# Autodesk Inventor assembly: assembly
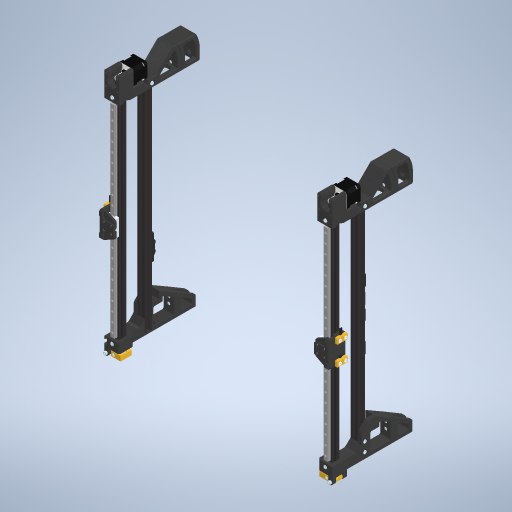
[picture p0: Inventor's stored thumbnail of the model, 512x512]
Saved by Autodesk Inventor 2024 (Build 280153020, 153B)
## iProperties
Created: 2023-11-07
Part Number: assembly
Description: FreeCAD Model
Document SubType Name: Assembly
Designer: torban
Authority: Unknown
Sending System: FreeCAD
Preprocessor: Open CASCADE STEP processor 7.6
Title: Open CASCADE Shape Model
Author: Author
## Documents named in this file (149)
- D:\GIT\lumenpnp\pnp\cad\STEP\Y-Gantry\Y-Gantry.iam
- D:\GIT\lumenpnp\pnp\cad\STEP\Y-Gantry\extrusion-cable-clip002.ipt
- D:\GIT\lumenpnp\pnp\cad\STEP\Y-Gantry\Y-Gantry-Left.iam
- D:\GIT\lumenpnp\pnp\cad\STEP\Y-Gantry\Back-Right-Leg.iam
- D:\GIT\lumenpnp\pnp\cad\STEP\Y-Gantry\Front-Right-Leg.iam
- D:\GIT\lumenpnp\pnp\cad\STEP\Y-Gantry\Y-Gantry-Right-Linear-Rail.iam
- D:\GIT\lumenpnp\pnp\cad\STEP\Y-Gantry\Y-Gantry-Slider-Right.iam
- D:\GIT\lumenpnp\pnp\cad\STEP\Y-Gantry\extrusion-cable-clip003.ipt
- D:\GIT\lumenpnp\pnp\cad\STEP\Y-Gantry\extrusion-cable-clip001.ipt
- D:\GIT\lumenpnp\pnp\cad\STEP\Y-Gantry\extrusion-cable-clip.ipt
- D:\GIT\lumenpnp\pnp\cad\STEP\Y-Gantry\vslot-extrusion-20mmx20mmx600mm001.ipt
- D:\GIT\lumenpnp\pnp\cad\STEP\Y-Gantry\vslot-extrusion-20mmx20mmx600mm002.ipt
- D:\GIT\lumenpnp\pnp\cad\STEP\Y-Gantry\GT2-pulley003.ipt
- D:\GIT\lumenpnp\pnp\cad\STEP\Y-Gantry\M3x8-Screw466.ipt
- D:\GIT\lumenpnp\pnp\cad\STEP\Y-Gantry\M3x8-Screw467.ipt
- D:\GIT\lumenpnp\pnp\cad\STEP\Y-Gantry\M3x8-Screw468.ipt
- D:\GIT\lumenpnp\pnp\cad\STEP\Y-Gantry\M3x8-Screw469.ipt
- D:\GIT\lumenpnp\pnp\cad\STEP\Y-Gantry\NEMA17-stepper004.ipt
- D:\GIT\lumenpnp\pnp\cad\STEP\Y-Gantry\M5x10-Screw345.ipt
- D:\GIT\lumenpnp\pnp\cad\STEP\Y-Gantry\M5x10-Screw346.ipt
- D:\GIT\lumenpnp\pnp\cad\STEP\Y-Gantry\M5x10-Screw347.ipt
- D:\GIT\lumenpnp\pnp\cad\STEP\Y-Gantry\M5-tslot-nut013.ipt
- D:\GIT\lumenpnp\pnp\cad\STEP\Y-Gantry\M5-tslot-nut014.ipt
- D:\GIT\lumenpnp\pnp\cad\STEP\Y-Gantry\M5-tslot-nut015.ipt
- D:\GIT\lumenpnp\pnp\cad\STEP\Y-Gantry\back-leg.ipt
- D:\GIT\lumenpnp\pnp\cad\STEP\Y-Gantry\Back-Right-Leg-Extension.iam
- D:\GIT\lumenpnp\pnp\cad\STEP\Y-Gantry\back-leg-extension_001.ipt
- D:\GIT\lumenpnp\pnp\cad\STEP\Y-Gantry\M5-Nut1086.ipt
- D:\GIT\lumenpnp\pnp\cad\STEP\Y-Gantry\M5x16-Screw219.ipt
- D:\GIT\lumenpnp\pnp\cad\STEP\Y-Gantry\M5-tslot-nut008.ipt
- D:\GIT\lumenpnp\pnp\cad\STEP\Y-Gantry\GT2-idler003.ipt
- D:\GIT\lumenpnp\pnp\cad\STEP\Y-Gantry\M5-Nut627.ipt
- D:\GIT\lumenpnp\pnp\cad\STEP\Y-Gantry\M5x25-Screw128.ipt
- D:\GIT\lumenpnp\pnp\cad\STEP\Y-Gantry\M5-Nut628.ipt
- D:\GIT\lumenpnp\pnp\cad\STEP\Y-Gantry\M3x16-Screw086.ipt
- D:\GIT\lumenpnp\pnp\cad\STEP\Y-Gantry\M3-Nut465.ipt
- D:\GIT\lumenpnp\pnp\cad\STEP\Y-Gantry\M5x10-Screw338.ipt
- D:\GIT\lumenpnp\pnp\cad\STEP\Y-Gantry\M5x10-Screw339.ipt
- D:\GIT\lumenpnp\pnp\cad\STEP\Y-Gantry\M5x10-Screw340.ipt
- D:\GIT\lumenpnp\pnp\cad\STEP\Y-Gantry\M5-tslot-nut007.ipt
- D:\GIT\lumenpnp\pnp\cad\STEP\Y-Gantry\M3-cap-nut.ipt
- D:\GIT\lumenpnp\pnp\cad\STEP\Y-Gantry\M5-tslot-nut009.ipt
- D:\GIT\lumenpnp\pnp\cad\STEP\Y-Gantry\M5x40-Screw345.ipt
- D:\GIT\lumenpnp\pnp\cad\STEP\Y-Gantry\y2-belt-tension-arm.ipt
- D:\GIT\lumenpnp\pnp\cad\STEP\Y-Gantry\front-right-leg.ipt
- D:\GIT\lumenpnp\pnp\cad\STEP\Y-Gantry\Front-Right-Leg-Extension.iam
- D:\GIT\lumenpnp\pnp\cad\STEP\Y-Gantry\M5x16-Screw222.ipt
- D:\GIT\lumenpnp\pnp\cad\STEP\Y-Gantry\M5x16-Screw221.ipt
- D:\GIT\lumenpnp\pnp\cad\STEP\Y-Gantry\front-leg-extension_001.ipt
- D:\GIT\lumenpnp\pnp\cad\STEP\Y-Gantry\M5-Nut1087.ipt
- D:\GIT\lumenpnp\pnp\cad\STEP\Y-Gantry\M5-Nut1088.ipt
- D:\GIT\lumenpnp\pnp\cad\STEP\Y-Gantry\Array002.iam
- D:\GIT\lumenpnp\pnp\cad\STEP\Y-Gantry\550mm-MGN12H001_002.ipt
- D:\GIT\lumenpnp\pnp\cad\STEP\Y-Gantry\m3_t-nut_bar-525mm.ipt
- D:\GIT\lumenpnp\pnp\cad\STEP\Y-Gantry\M3x8-Screw814.ipt
- D:\GIT\lumenpnp\pnp\cad\STEP\Y-Gantry\M5x10-Screw595.ipt
- D:\GIT\lumenpnp\pnp\cad\STEP\Y-Gantry\M5x10-Screw596.ipt
- D:\GIT\lumenpnp\pnp\cad\STEP\Y-Gantry\y-gantry_005.ipt
- D:\GIT\lumenpnp\pnp\cad\STEP\Y-Gantry\M5x10-Screw597.ipt
- D:\GIT\lumenpnp\pnp\cad\STEP\Y-Gantry\M5x10-Screw598.ipt
- D:\GIT\lumenpnp\pnp\cad\STEP\Y-Gantry\M5-Nut1019.ipt
- D:\GIT\lumenpnp\pnp\cad\STEP\Y-Gantry\belt-clamp013.ipt
- D:\GIT\lumenpnp\pnp\cad\STEP\Y-Gantry\M3x8-Screw961.ipt
- D:\GIT\lumenpnp\pnp\cad\STEP\Y-Gantry\M3x8-Screw962.ipt
- D:\GIT\lumenpnp\pnp\cad\STEP\Y-Gantry\M3x8-Screw963.ipt
- D:\GIT\lumenpnp\pnp\cad\STEP\Y-Gantry\belt-clamp014.ipt
- D:\GIT\lumenpnp\pnp\cad\STEP\Y-Gantry\MGN12H001_004.ipt
- D:\GIT\lumenpnp\pnp\cad\STEP\Y-Gantry\M3x8-Screw827.ipt
- D:\GIT\lumenpnp\pnp\cad\STEP\Y-Gantry\M5-Nut1022.ipt
- D:\GIT\lumenpnp\pnp\cad\STEP\Y-Gantry\M5-Nut1023.ipt
- D:\GIT\lumenpnp\pnp\cad\STEP\Y-Gantry\M5-Nut1030.ipt
- D:\GIT\lumenpnp\pnp\cad\STEP\Y-Gantry\M5-Nut1028.ipt
- D:\GIT\lumenpnp\pnp\cad\STEP\Y-Gantry\M5-Nut1029.ipt
- D:\GIT\lumenpnp\pnp\cad\STEP\Y-Gantry\y-gantry-gt2-belt_right.ipt
- D:\GIT\lumenpnp\pnp\cad\STEP\Y-Gantry\Y-Left-Extrusion.iam
- D:\GIT\lumenpnp\pnp\cad\STEP\Y-Gantry\Back-Left-Leg.iam
- D:\GIT\lumenpnp\pnp\cad\STEP\Y-Gantry\Front-Left-Leg.iam
- D:\GIT\lumenpnp\pnp\cad\STEP\Y-Gantry\Y-Gantry-Left-Linear-Rail.iam
- D:\GIT\lumenpnp\pnp\cad\STEP\Y-Gantry\Y-Gantry-Slider-Left.iam
- D:\GIT\lumenpnp\pnp\cad\STEP\Y-Gantry\umbilical-cable-strain-relief.ipt
- D:\GIT\lumenpnp\pnp\cad\STEP\Y-Gantry\vslot-extrusion-20mmx20mmx600mm.ipt
- D:\GIT\lumenpnp\pnp\cad\STEP\Y-Gantry\M5x10-Screw349.ipt
- D:\GIT\lumenpnp\pnp\cad\STEP\Y-Gantry\M5x10-Screw348.ipt
- D:\GIT\lumenpnp\pnp\cad\STEP\Y-Gantry\M5-tslot-nut016.ipt
- D:\GIT\lumenpnp\pnp\cad\STEP\Y-Gantry\M5-tslot-nut017.ipt
- D:\GIT\lumenpnp\pnp\cad\STEP\Y-Gantry\vslot-extrusion-20mmx20mmx600mm003.ipt
- D:\GIT\lumenpnp\pnp\cad\STEP\Y-Gantry\M3x8-Screw462.ipt
- D:\GIT\lumenpnp\pnp\cad\STEP\Y-Gantry\M3x8-Screw463.ipt
- D:\GIT\lumenpnp\pnp\cad\STEP\Y-Gantry\M3x8-Screw464.ipt
- D:\GIT\lumenpnp\pnp\cad\STEP\Y-Gantry\M3x8-Screw465.ipt
- D:\GIT\lumenpnp\pnp\cad\STEP\Y-Gantry\NEMA17-stepper003.ipt
- D:\GIT\lumenpnp\pnp\cad\STEP\Y-Gantry\GT2-pulley002.ipt
- D:\GIT\lumenpnp\pnp\cad\STEP\Y-Gantry\M5x10-Screw342.ipt
- D:\GIT\lumenpnp\pnp\cad\STEP\Y-Gantry\M5x10-Screw343.ipt
- D:\GIT\lumenpnp\pnp\cad\STEP\Y-Gantry\M5x10-Screw344.ipt
- D:\GIT\lumenpnp\pnp\cad\STEP\Y-Gantry\M5-tslot-nut010.ipt
- D:\GIT\lumenpnp\pnp\cad\STEP\Y-Gantry\M5-tslot-nut011.ipt
- D:\GIT\lumenpnp\pnp\cad\STEP\Y-Gantry\M5-tslot-nut012.ipt
- D:\GIT\lumenpnp\pnp\cad\STEP\Y-Gantry\back-leg001.ipt
- D:\GIT\lumenpnp\pnp\cad\STEP\Y-Gantry\Back-Left-Leg-Extension.iam
- D:\GIT\lumenpnp\pnp\cad\STEP\Y-Gantry\M5-Nut1085.ipt
- D:\GIT\lumenpnp\pnp\cad\STEP\Y-Gantry\back-leg-extension_002.ipt
- D:\GIT\lumenpnp\pnp\cad\STEP\Y-Gantry\M5x16-Screw220.ipt
- D:\GIT\lumenpnp\pnp\cad\STEP\Y-Gantry\M5-tslot-nut002.ipt
- D:\GIT\lumenpnp\pnp\cad\STEP\Y-Gantry\M3-Nut464.ipt
- D:\GIT\lumenpnp\pnp\cad\STEP\Y-Gantry\M5-Nut625.ipt
- D:\GIT\lumenpnp\pnp\cad\STEP\Y-Gantry\GT2-idler002.ipt
- D:\GIT\lumenpnp\pnp\cad\STEP\Y-Gantry\M5-Nut626.ipt
- D:\GIT\lumenpnp\pnp\cad\STEP\Y-Gantry\M3x16-Screw085.ipt
- D:\GIT\lumenpnp\pnp\cad\STEP\Y-Gantry\M5x10-Screw334.ipt
- D:\GIT\lumenpnp\pnp\cad\STEP\Y-Gantry\M5x25-Screw127.ipt
- D:\GIT\lumenpnp\pnp\cad\STEP\Y-Gantry\M5x10-Screw335.ipt
- D:\GIT\lumenpnp\pnp\cad\STEP\Y-Gantry\M5x10-Screw336.ipt
- D:\GIT\lumenpnp\pnp\cad\STEP\Y-Gantry\M5x40-Screw344.ipt
- D:\GIT\lumenpnp\pnp\cad\STEP\Y-Gantry\M5-tslot-nut003.ipt
- D:\GIT\lumenpnp\pnp\cad\STEP\Y-Gantry\M5-tslot-nut004.ipt
- D:\GIT\lumenpnp\pnp\cad\STEP\Y-Gantry\front-left-leg.ipt
- D:\GIT\lumenpnp\pnp\cad\STEP\Y-Gantry\M3-cap-nut002.ipt
- D:\GIT\lumenpnp\pnp\cad\STEP\Y-Gantry\y1-belt-tension-arm.ipt
- D:\GIT\lumenpnp\pnp\cad\STEP\Y-Gantry\M5-Nut663.ipt
- D:\GIT\lumenpnp\pnp\cad\STEP\Y-Gantry\Front-Left-Leg-Extension.iam
- D:\GIT\lumenpnp\pnp\cad\STEP\Y-Gantry\M5x16-Screw228.ipt
- D:\GIT\lumenpnp\pnp\cad\STEP\Y-Gantry\M5-Nut1094.ipt
- D:\GIT\lumenpnp\pnp\cad\STEP\Y-Gantry\M5-Nut1093.ipt
- D:\GIT\lumenpnp\pnp\cad\STEP\Y-Gantry\front-leg-extension_002.ipt
- D:\GIT\lumenpnp\pnp\cad\STEP\Y-Gantry\M5x16-Screw227.ipt
- D:\GIT\lumenpnp\pnp\cad\STEP\Y-Gantry\Array.iam
- D:\GIT\lumenpnp\pnp\cad\STEP\Y-Gantry\550mm-MGN12H001_001.ipt
- D:\GIT\lumenpnp\pnp\cad\STEP\Y-Gantry\m3_t-nut_bar-525mm002.ipt
- D:\GIT\lumenpnp\pnp\cad\STEP\Y-Gantry\M3x8-Screw815.ipt
- D:\GIT\lumenpnp\pnp\cad\STEP\Y-Gantry\M5x10-Screw591.ipt
- D:\GIT\lumenpnp\pnp\cad\STEP\Y-Gantry\M5x10-Screw592.ipt
- D:\GIT\lumenpnp\pnp\cad\STEP\Y-Gantry\y-gantry_003.ipt
- D:\GIT\lumenpnp\pnp\cad\STEP\Y-Gantry\M5x10-Screw593.ipt
- D:\GIT\lumenpnp\pnp\cad\STEP\Y-Gantry\M5x10-Screw594.ipt
- D:\GIT\lumenpnp\pnp\cad\STEP\Y-Gantry\M5-Nut1008.ipt
- D:\GIT\lumenpnp\pnp\cad\STEP\Y-Gantry\M5-Nut1006.ipt
- D:\GIT\lumenpnp\pnp\cad\STEP\Y-Gantry\M5-Nut1013.ipt
- D:\GIT\lumenpnp\pnp\cad\STEP\Y-Gantry\M5-Nut1007.ipt
- D:\GIT\lumenpnp\pnp\cad\STEP\Y-Gantry\belt-clamp009.ipt
- D:\GIT\lumenpnp\pnp\cad\STEP\Y-Gantry\M3x8-Screw958.ipt
- D:\GIT\lumenpnp\pnp\cad\STEP\Y-Gantry\M3x8-Screw959.ipt
- D:\GIT\lumenpnp\pnp\cad\STEP\Y-Gantry\M3x8-Screw960.ipt
- D:\GIT\lumenpnp\pnp\cad\STEP\Y-Gantry\belt-clamp010.ipt
- D:\GIT\lumenpnp\pnp\cad\STEP\Y-Gantry\M3x8-Screw823.ipt
- D:\GIT\lumenpnp\pnp\cad\STEP\Y-Gantry\MGN12H001_001.ipt
- D:\GIT\lumenpnp\pnp\cad\STEP\Y-Gantry\M5-Nut1009.ipt
- D:\GIT\lumenpnp\pnp\cad\STEP\Y-Gantry\M5-Nut1014.ipt
- D:\GIT\lumenpnp\pnp\cad\STEP\Y-Gantry\y-gantry-gt2-belt_left.ipt
## Components (148 placed, 148 different names)
1. 3662
2. 3749 [sub-assembly] — Flush:1
3. 3767 [sub-assembly]
4. 3790 [sub-assembly]
5. 3806 [sub-assembly]
6. 3826 [sub-assembly] — Flush:1
7. 3827
8. 3828
9. 3829
10. 3830
11. 3831
12. 3832
13. 3833
14. 3834
15. 3835
16. 3836
17. 3837
18. 3838
19. 3839
20. 3840
21. 3841
22. 3842
23. 3843
24. 3844
25. 3845 [sub-assembly]
26. 3846
27. 3847
28. 3848
29. 3849
30. 3850
31. 3851
32. 3852
33. 3853
34. 3854
35. 3855
36. 3856
37. 3857
38. 3858
39. 3859
40. 3860
41. 3861
42. 3862
43. 3863
44. 3864
45. 3865 [sub-assembly]
46. 3866
47. 3867
48. 3868
49. 3869
50. 3870
51. 3871 [sub-assembly]
52. 3872
53. 3873
54. 3874
55. 3875
56. 3876
57. 3877
58. 3878
59. 3879
60. 3880
61. 3881
62. 3882
63. 3883
64. 3884
65. 3885
66. 3886
67. 3887
68. 3888
69. 3889
70. 3890
71. 3891
72. 3892
73. 3893
74. 3894 [sub-assembly]
75. 3895 [sub-assembly]
76. 3896 [sub-assembly]
77. 3897 [sub-assembly]
78. 3898 [sub-assembly]
79. 3899
80. 3900
81. 3901
82. 3902
83. 3903
84. 3904
85. 3905
86. 3906
87. 3907
88. 3908
89. 3909
90. 3910
91. 3911
92. 3912
93. 3913
94. 3914
95. 3915
96. 3916
97. 3917
98. 3918
99. 3919 [sub-assembly]
100. 3920
101. 3921
102. 3922
103. 3923
104. 3924
105. 3925
106. 3926
107. 3927
108. 3928
109. 3929
110. 3930
111. 3931
112. 3932
113. 3933
114. 3934
115. 3935
116. 3936
117. 3937
118. 3938
119. 3939
120. 3940 [sub-assembly]
121. 3941
122. 3942
123. 3943
124. 3944
125. 3945
126. 3946 [sub-assembly]
127. 3947
128. 3948
129. 3949
130. 3950
131. 3951
132. 3952
133. 3953
134. 3954
135. 3955
136. 3956
137. 3957
138. 3958
139. 3959
140. 3960
141. 3961
142. 3962
143. 3963
144. 3964
145. 3965
146. 3966
147. 3967
148. 3968
## Relationships (1: Flush 1)
- Flush:1: 3749 ↔ 3826
